# Autodesk Inventor assembly: Tower Bridge Assembly
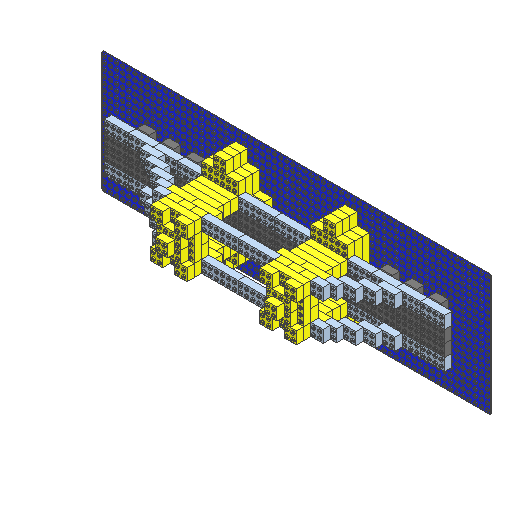
[picture p0: Inventor's stored thumbnail of the model, 512x512]
Saved by Autodesk Inventor 2026.2 (Build 302298000, 298)
## iProperties
Created: 2026-01-06
Part Number: Tower Bridge Assembly
Document SubType Name: Assembly
Designer: andyeske
Author: andyeske
## Documents named in this file (6)
- C:\Users\andyeske\Inventor\Tower Bridge Assembly.iam
- C:\Users\andyeske\Inventor\LEGO 2x4 Brick.ipt
- C:\Users\andyeske\Inventor\LEGO 2x6 Brick.ipt
- C:\Users\andyeske\Inventor\LEGO 2x2 Brick.ipt
- C:\Users\andyeske\Inventor\LEGO 2x3 Brick.ipt
- C:\Users\andyeske\Inventor\LEGO 20x64 Plate.ipt
## Components (185 placed, 5 different names)
1. LEGO 20x64 Plate:1 — Mate:33, Flush:46
2. LEGO 2x2 Brick:13 — Mate:22, Flush:32, Flush:33
3. LEGO 2x2 Brick:18
4. LEGO 2x4 Brick:18 — Mate:12, Flush:17, Flush:18, Mate:13, Cylindrical:4, Mate:14, Flush:21, Mate:25, Flush:35
5. LEGO 2x4 Brick:17 — Mate:12, Flush:17, Flush:18, Flush:19, Flush:20, Flush:44, Flush:45
6. LEGO 2x6 Brick:21 — Mate:15, Flush:22, Flush:23, Mate:16, Flush:24, Flush:25, Flush:36
7. LEGO 2x4 Brick:22
8. LEGO 2x4 Brick:23
9. LEGO 2x6 Brick:31
10. LEGO 2x6 Brick:39 — Flush:44, Mate:31, Flush:45
11. LEGO 2x6 Brick:40
12. LEGO 2x6 Brick:7 — Mate:32
13. LEGO 2x6 Brick:38
14. LEGO 2x6 Brick:6 — Mate:8, Flush:13, Flush:14, Flush:43, Mate:29
15. LEGO 2x6 Brick:37
16. LEGO 2x6 Brick:5 — Mate:5, Flush:7, Flush:8, Mate:9
17. LEGO 2x6 Brick:16
18. LEGO 2x6 Brick:17
19. LEGO 2x6 Brick:4 — Mate:5, Flush:7, Flush:8, Mate:6, Flush:9, Flush:10, Mate:8, Flush:13, Flush:14, Cylindrical:3
20. LEGO 2x6 Brick:14 — Mate:11, Flush:15
21. LEGO 2x6 Brick:15 — Flush:16
22. LEGO 2x2 Brick:3 — Mate:17, Flush:26, Flush:27
23. LEGO 2x2 Brick:4
24. LEGO 2x2 Brick:5 — Flush:46
25. LEGO 2x2 Brick:6
26. LEGO 2x2 Brick:7
27. LEGO 2x2 Brick:8
28. LEGO 2x6 Brick:35 — Flush:43, Mate:29, Mate:30
29. LEGO 2x6 Brick:36
30. LEGO 2x4 Brick:1 — Mate:1, Flush:1, Flush:2, Cylindrical:2
31. LEGO 2x4 Brick:2 — Mate:1, Flush:1, Flush:2, Mate:3, Flush:5, Flush:6
32. LEGO 2x4 Brick:3 — Mate:3, Flush:5, Flush:6
33. LEGO 2x4 Brick:4
34. LEGO 2x4 Brick:5
35. LEGO 2x4 Brick:6
36. LEGO 2x4 Brick:7
37. LEGO 2x4 Brick:8
38. LEGO 2x4 Brick:9
39. LEGO 2x4 Brick:10 — Mate:4
40. LEGO 2x4 Brick:11
41. LEGO 2x4 Brick:12 — Mate:6, Flush:9
42. LEGO 2x4 Brick:13 — Cylindrical:1
43. LEGO 2x4 Brick:14
44. LEGO 2x4 Brick:15
45. LEGO 2x4 Brick:16 — Flush:10, Mate:10
46. LEGO 2x3 Brick:3 — Flush:39, Mate:27, Flush:40
47. LEGO 2x3 Brick:2 — Flush:37, Flush:38, Mate:26, Flush:39, Mate:27, Flush:40
48. LEGO 2x3 Brick:1 — Flush:37, Flush:38, Mate:26, Mate:28, Flush:41, Flush:42
49. LEGO 2x2 Brick:15 — Mate:23, Flush:34, Mate:24, Mate:28, Flush:41, Flush:42
50. LEGO 2x2 Brick:14 — Mate:23, Flush:34, Mate:24, Mate:25, Flush:35, Flush:36
51. LEGO 2x3 Brick:4
52. LEGO 2x3 Brick:5
53. LEGO 2x3 Brick:6
54. LEGO 2x2 Brick:16
55. LEGO 2x2 Brick:17
56. LEGO 2x4 Brick:30 — Mate:20, Flush:31, Mate:21, Mate:22, Flush:32, Flush:33
57. LEGO 2x4 Brick:31
58. LEGO 2x4 Brick:27 — Cylindrical:5, Mate:19, Flush:30, Mate:20, Flush:31
59. LEGO 2x4 Brick:28
60. LEGO 2x4 Brick:29
61. LEGO 2x4 Brick:38
62. LEGO 2x4 Brick:39
63. LEGO 2x6 Brick:41
64. LEGO 2x4 Brick:40
65. LEGO 2x4 Brick:41
66. LEGO 2x6 Brick:45
67. LEGO 2x6 Brick:49
68. LEGO 2x6 Brick:50
69. LEGO 2x6 Brick:51
70. LEGO 2x6 Brick:52
71. LEGO 2x6 Brick:53
72. LEGO 2x6 Brick:54
73. LEGO 2x6 Brick:55
74. LEGO 2x6 Brick:56
75. LEGO 2x6 Brick:57
76. LEGO 2x6 Brick:58
77. LEGO 2x6 Brick:59
78. LEGO 2x6 Brick:60
79. LEGO 2x2 Brick:23
80. LEGO 2x2 Brick:24 — Mate:33
81. LEGO 2x2 Brick:25
82. LEGO 2x2 Brick:26
83. LEGO 2x2 Brick:27
84. LEGO 2x2 Brick:28
85. LEGO 2x6 Brick:79
86. LEGO 2x6 Brick:80
87. LEGO 2x4 Brick:42
88. LEGO 2x4 Brick:43
89. LEGO 2x4 Brick:44
90. LEGO 2x4 Brick:45
91. LEGO 2x4 Brick:46
92. LEGO 2x4 Brick:47
93. LEGO 2x4 Brick:48
94. LEGO 2x4 Brick:49
95. LEGO 2x4 Brick:50
96. LEGO 2x4 Brick:51
97. LEGO 2x4 Brick:52
98. LEGO 2x4 Brick:53
99. LEGO 2x4 Brick:54
100. LEGO 2x4 Brick:55
101. LEGO 2x4 Brick:56
102. LEGO 2x4 Brick:57
103. LEGO 2x3 Brick:7
104. LEGO 2x3 Brick:8
105. LEGO 2x3 Brick:9
106. LEGO 2x2 Brick:29
107. LEGO 2x2 Brick:30
108. LEGO 2x3 Brick:10
109. LEGO 2x3 Brick:11
110. LEGO 2x3 Brick:12
111. LEGO 2x2 Brick:31
112. LEGO 2x2 Brick:32
113. LEGO 2x4 Brick:58
114. LEGO 2x4 Brick:59
115. LEGO 2x4 Brick:60
116. LEGO 2x4 Brick:61
117. LEGO 2x4 Brick:62
118. LEGO 2x4 Brick:19 — Cylindrical:4, Mate:14, Flush:21, Mate:15, Flush:22, Cylindrical:5
119. LEGO 2x4 Brick:20
120. LEGO 2x4 Brick:21 — Flush:23, Mate:31
121. LEGO 2x4 Brick:24 — Mate:19, Flush:30
122. LEGO 2x4 Brick:25
123. LEGO 2x4 Brick:26
124. LEGO 2x6 Brick:18 — Mate:11, Flush:15, Flush:16
125. LEGO 2x6 Brick:19
126. LEGO 2x6 Brick:20 — Mate:13, Flush:19, Flush:20
127. LEGO 2x2 Brick:1 — Mate:16, Flush:24, Flush:25
128. LEGO 2x2 Brick:2
129. LEGO 2x6 Brick:32
130. LEGO 2x6 Brick:33
131. LEGO 2x6 Brick:34
132. LEGO 2x2 Brick:9 — Mate:21
133. LEGO 2x2 Brick:10
134. LEGO 2x6 Brick:1 — Cylindrical:1, Mate:4, Cylindrical:2
135. LEGO 2x6 Brick:2
136. LEGO 2x6 Brick:3
137. LEGO 2x6 Brick:8 — Cylindrical:3, Mate:9, Mate:10
138. LEGO 2x6 Brick:9
139. LEGO 2x6 Brick:10
140. LEGO 2x6 Brick:11
141. LEGO 2x6 Brick:12 — Mate:30
142. LEGO 2x6 Brick:13
143. LEGO 2x6 Brick:22
144. LEGO 2x6 Brick:23
145. LEGO 2x6 Brick:24
146. LEGO 2x6 Brick:25 — Flush:27
147. LEGO 2x6 Brick:26
148. LEGO 2x6 Brick:27 — Mate:17, Flush:26
149. LEGO 2x6 Brick:28
150. LEGO 2x6 Brick:29
151. LEGO 2x6 Brick:30
152. LEGO 2x4 Brick:32
153. LEGO 2x4 Brick:33
154. LEGO 2x4 Brick:34
155. LEGO 2x4 Brick:35
156. LEGO 2x4 Brick:36
157. LEGO 2x4 Brick:37
158. LEGO 2x6 Brick:42
159. LEGO 2x6 Brick:43
160. LEGO 2x6 Brick:44
161. LEGO 2x2 Brick:19
162. LEGO 2x2 Brick:20
163. LEGO 2x6 Brick:46
164. LEGO 2x6 Brick:47
165. LEGO 2x6 Brick:48
166. LEGO 2x2 Brick:21
167. LEGO 2x2 Brick:22
168. LEGO 2x6 Brick:61
169. LEGO 2x6 Brick:62
170. LEGO 2x6 Brick:63
171. LEGO 2x6 Brick:64
172. LEGO 2x6 Brick:65
173. LEGO 2x6 Brick:66
174. LEGO 2x6 Brick:67
175. LEGO 2x6 Brick:68
176. LEGO 2x6 Brick:69
177. LEGO 2x6 Brick:70
178. LEGO 2x6 Brick:71
179. LEGO 2x6 Brick:72
180. LEGO 2x6 Brick:73
181. LEGO 2x6 Brick:74
182. LEGO 2x6 Brick:75
183. LEGO 2x6 Brick:76
184. LEGO 2x6 Brick:77
185. LEGO 2x6 Brick:78
## Component patterns: (2 elements, first: LEGO 2x2 Brick:13), (2 elements), (2 elements, first: LEGO 2x4 Brick:18 + LEGO 2x4 Brick:17 + LEGO 2x6 Brick:21), (2 elements, first: LEGO 2x6 Brick:39), (2 elements, first: LEGO 2x6 Brick:7), (2 elements, first: LEGO 2x6 Brick:6), (3 elements, first: LEGO 2x6 Brick:5), (3 elements, first: LEGO 2x6 Brick:4), (2 elements), (6 elements, first: LEGO 2x2 Brick:3), (2 elements, first: LEGO 2x6 Brick:35), (4 elements, first: LEGO 2x4 Brick:1 + LEGO 2x4 Brick:2 + LEGO 2x4 Brick:3 + LEGO 2x4 Brick:4), (2 elements, first: LEGO 2x3 Brick:3 + LEGO 2x3 Brick:2 + LEGO 2x3 Brick:1 + LEGO 2x2 Brick:15 + LEGO 2x2 Brick:14), (2 elements, first: LEGO 2x4 Brick:30), (3 elements, first: LEGO 2x4 Brick:27), Component Pattern 12:2 (2 elements), Component Pattern 11:2 (2 elements), Component Pattern 20:2 (2 elements), Component Pattern 19:2 (2 elements), Component Pattern 18:2 (2 elements), Component Pattern 5:2 (3 elements), Component Pattern 4:2 (3 elements), Component Pattern 9:2 (2 elements), Component Pattern 10:2 (6 elements), Component Pattern 17:2 (2 elements), Component Pattern 1:2 (4 elements), Component Pattern 16:2 (2 elements), Component Pattern 15:2 (2 elements), Component Pattern 14:2 (3 elements), (3 elements, first: LEGO 2x4 Brick:19), Component Pattern 7:2 (3 elements), (3 elements, first: LEGO 2x6 Brick:18), (2 elements, first: LEGO 2x2 Brick:1), Component Pattern 6:2 (3 elements), Component Pattern 8:2 (2 elements), (3 elements, first: LEGO 2x6 Brick:1), (6 elements, first: LEGO 2x6 Brick:8), Component Pattern 2:2 (3 elements), Component Pattern 3:2 (6 elements), Component Pattern 7:3 (3 elements), Component Pattern 7:4 (3 elements), Component Pattern 6:3 (3 elements), Component Pattern 8:3 (2 elements), Component Pattern 6:4 (3 elements), Component Pattern 8:4 (2 elements), Component Pattern 2:3 (3 elements), Component Pattern 3:3 (6 elements), Component Pattern 2:4 (3 elements), Component Pattern 3:4 (6 elements)
## Relationships (81: Flush 44, Mate 32, CylindricalJoint 5)
- Mate:1: LEGO 2x4 Brick:1 ↔ LEGO 2x4 Brick:2
- Flush:1: LEGO 2x4 Brick:1 ↔ LEGO 2x4 Brick:2
- Flush:2: LEGO 2x4 Brick:1 ↔ LEGO 2x4 Brick:2
- [Mate]: LEGO 2x4 Brick:3 ↔ LEGO 2x4 Brick:4
- [Flush]: LEGO 2x4 Brick:3 ↔ LEGO 2x4 Brick:4
- [Flush]: LEGO 2x4 Brick:3 ↔ LEGO 2x4 Brick:4
- Mate:3: LEGO 2x4 Brick:2 ↔ LEGO 2x4 Brick:3
- Flush:5: LEGO 2x4 Brick:2 ↔ LEGO 2x4 Brick:3
- Flush:6: LEGO 2x4 Brick:2 ↔ LEGO 2x4 Brick:3
- Cylindrical:1: LEGO 2x4 Brick:13 ↔ LEGO 2x6 Brick:1
- Mate:4: LEGO 2x4 Brick:10 ↔ LEGO 2x6 Brick:1
- Cylindrical:2: LEGO 2x4 Brick:1 ↔ LEGO 2x6 Brick:1
- Mate:5: LEGO 2x6 Brick:5 ↔ LEGO 2x6 Brick:4
- Flush:7: LEGO 2x6 Brick:5 ↔ LEGO 2x6 Brick:4
- Flush:8: LEGO 2x6 Brick:5 ↔ LEGO 2x6 Brick:4
- Mate:6: LEGO 2x6 Brick:4 ↔ LEGO 2x4 Brick:12
- Flush:9: LEGO 2x6 Brick:4 ↔ LEGO 2x4 Brick:12
- Flush:10 (16 mm): LEGO 2x6 Brick:4 ↔ LEGO 2x4 Brick:16
- [Mate]: LEGO 2x6 Brick:7 ↔ LEGO 2x6 Brick:6
- [Flush]: LEGO 2x6 Brick:7 ↔ LEGO 2x6 Brick:6
- [Flush]: LEGO 2x6 Brick:7 ↔ LEGO 2x6 Brick:6
- Mate:8: LEGO 2x6 Brick:6 ↔ LEGO 2x6 Brick:4
- Flush:13: LEGO 2x6 Brick:6 ↔ LEGO 2x6 Brick:4
- Flush:14: LEGO 2x6 Brick:6 ↔ LEGO 2x6 Brick:4
- Cylindrical:3: LEGO 2x6 Brick:4 ↔ LEGO 2x6 Brick:8
- Mate:9: LEGO 2x6 Brick:5 ↔ LEGO 2x6 Brick:8
- Mate:10: LEGO 2x4 Brick:16 ↔ LEGO 2x6 Brick:8
- Mate:11: LEGO 2x6 Brick:14 ↔ LEGO 2x6 Brick:18
- Flush:15: LEGO 2x6 Brick:14 ↔ LEGO 2x6 Brick:18
- Flush:16 (16 mm): LEGO 2x6 Brick:15 ↔ LEGO 2x6 Brick:18
- Mate:12: LEGO 2x4 Brick:18 ↔ LEGO 2x4 Brick:17
- Flush:17: LEGO 2x4 Brick:18 ↔ LEGO 2x4 Brick:17
- Flush:18: LEGO 2x4 Brick:18 ↔ LEGO 2x4 Brick:17
- Mate:13: LEGO 2x4 Brick:18 ↔ LEGO 2x6 Brick:20
- Flush:19 (-8 mm): LEGO 2x4 Brick:17 ↔ LEGO 2x6 Brick:20
- Flush:20: LEGO 2x4 Brick:17 ↔ LEGO 2x6 Brick:20
- Cylindrical:4: LEGO 2x4 Brick:18 ↔ LEGO 2x4 Brick:19
- Mate:14: LEGO 2x4 Brick:18 ↔ LEGO 2x4 Brick:19
- Flush:21: LEGO 2x4 Brick:18 ↔ LEGO 2x4 Brick:19
- Mate:15: LEGO 2x6 Brick:21 ↔ LEGO 2x4 Brick:19
- Flush:22: LEGO 2x6 Brick:21 ↔ LEGO 2x4 Brick:19
- Flush:23: LEGO 2x6 Brick:21 ↔ LEGO 2x4 Brick:21
- Mate:16: LEGO 2x6 Brick:21 ↔ LEGO 2x2 Brick:1
- Flush:24: LEGO 2x6 Brick:21 ↔ LEGO 2x2 Brick:1
- Flush:25: LEGO 2x6 Brick:21 ↔ LEGO 2x2 Brick:1
- Mate:17: LEGO 2x2 Brick:3 ↔ LEGO 2x6 Brick:27
- Flush:26: LEGO 2x2 Brick:3 ↔ LEGO 2x6 Brick:27
- Flush:27 (16 mm): LEGO 2x2 Brick:3 ↔ LEGO 2x6 Brick:25
- Cylindrical:5: LEGO 2x4 Brick:27 ↔ LEGO 2x4 Brick:19
- Mate:19: LEGO 2x4 Brick:27 ↔ LEGO 2x4 Brick:24
- Flush:30: LEGO 2x4 Brick:27 ↔ LEGO 2x4 Brick:24
- Mate:20: LEGO 2x4 Brick:30 ↔ LEGO 2x4 Brick:27
- Flush:31 (8 mm): LEGO 2x4 Brick:30 ↔ LEGO 2x4 Brick:27
- Mate:21: LEGO 2x4 Brick:30 ↔ LEGO 2x2 Brick:9
- Mate:22: LEGO 2x2 Brick:13 ↔ LEGO 2x4 Brick:30
- Flush:32 (8 mm): LEGO 2x2 Brick:13 ↔ LEGO 2x4 Brick:30
- Flush:33 (8 mm): LEGO 2x2 Brick:13 ↔ LEGO 2x4 Brick:30
- Mate:23 (-8 mm): LEGO 2x2 Brick:15 ↔ LEGO 2x2 Brick:14
- Flush:34: LEGO 2x2 Brick:15 ↔ LEGO 2x2 Brick:14
- Mate:24: LEGO 2x2 Brick:15 ↔ LEGO 2x2 Brick:14
- Mate:25: LEGO 2x4 Brick:18 ↔ LEGO 2x2 Brick:14
- Flush:35: LEGO 2x4 Brick:18 ↔ LEGO 2x2 Brick:14
- Flush:36 (-16 mm): LEGO 2x6 Brick:21 ↔ LEGO 2x2 Brick:14
- Flush:37: LEGO 2x3 Brick:2 ↔ LEGO 2x3 Brick:1
- Flush:38 (16 mm): LEGO 2x3 Brick:2 ↔ LEGO 2x3 Brick:1
- Mate:26: LEGO 2x3 Brick:2 ↔ LEGO 2x3 Brick:1
- Flush:39: LEGO 2x3 Brick:3 ↔ LEGO 2x3 Brick:2
- Mate:27: LEGO 2x3 Brick:3 ↔ LEGO 2x3 Brick:2
- Flush:40 (16 mm): LEGO 2x3 Brick:3 ↔ LEGO 2x3 Brick:2
- Mate:28: LEGO 2x3 Brick:1 ↔ LEGO 2x2 Brick:15
- Flush:41: LEGO 2x3 Brick:1 ↔ LEGO 2x2 Brick:15
- Flush:42 (16 mm): LEGO 2x3 Brick:1 ↔ LEGO 2x2 Brick:15
- Flush:43 (-8 mm): LEGO 2x6 Brick:6 ↔ LEGO 2x6 Brick:35
- Mate:29: LEGO 2x6 Brick:6 ↔ LEGO 2x6 Brick:35
- Mate:30: LEGO 2x6 Brick:35 ↔ LEGO 2x6 Brick:12
- Flush:44: LEGO 2x4 Brick:17 ↔ LEGO 2x6 Brick:39
- Mate:31: LEGO 2x6 Brick:39 ↔ LEGO 2x4 Brick:21
- Flush:45 (9.6 mm): LEGO 2x4 Brick:17 ↔ LEGO 2x6 Brick:39
- Mate:32: LEGO 2x6 Brick:7
- Mate:33: LEGO 20x64 Plate:1 ↔ LEGO 2x2 Brick:24
- Flush:46 (16 mm): LEGO 20x64 Plate:1 ↔ LEGO 2x2 Brick:5
## Named parameters: d3_d2 = 0 mm, d4_d0 = 0 mm, d5_d1 = 0 mm, d29_d22 = 0 mm, d30_d23 = 0 mm, d31_d24 = 0 mm, Finish10_Area = 38.2567, Finish11_Area = 870.442, Finish12_Area = 787.101, Finish13_Area = 1885.19, Finish14_Area = 1955.01, Finish1_Area = 306.053, Finish2_Area = 306.053, Finish3_Area = 169.316, Finish4_Area = 481.047, Finish5_Area = 395.072, Finish6_Area = 112.878, Finish7_Area = 892.409, Finish8_Area = 841.647, Finish9_Area = 225.755
note: some values were not read from the file. Shown as the stored number, unit unknown: "Finish10_Area", "Finish11_Area", "Finish12_Area", "Finish13_Area", "Finish14_Area", "Finish1_Area", "Finish2_Area", "Finish3_Area", "Finish4_Area", "Finish5_Area", "Finish6_Area", "Finish7_Area", "Finish8_Area", "Finish9_Area".
